# Autodesk Inventor assembly: Outer Shield
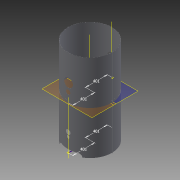
[picture p0: Inventor's stored thumbnail of the model, 180x180]
Saved by Autodesk Inventor 2015 (Build 190159000, 159)
## iProperties
Created: 2014-06-19
Part Number: Outer Shield
Document SubType Name: Assembly
Designer: Aki
Author: Aki
## Documents named in this file (6)
- C:\ColdMatter\CADFiles\EDM Machine\EDM Outer Shield\Outer Shield.iam
- C:\ColdMatter\CADFiles\EDM Machine\EDM Outer Shield\Lower Front Half.ipt
- C:\ColdMatter\CADFiles\EDM Machine\EDM Outer Shield\Lower Back Half.ipt
- C:\ColdMatter\CADFiles\EDM Machine\EDM Outer Shield\Upper Front Half.ipt
- C:\ColdMatter\CADFiles\EDM Machine\EDM Outer Shield\Upper Back Half.ipt
- C:\ColdMatter\CADFiles\EDM Machine\EDM Outer Shield\Band.ipt
## Components (6 placed, 5 different names)
1. Lower Front Half:1 — Mate:1, Mate:2, Mate:3, Mate:4, Mate:5, Mate:7
2. Lower Back Half:1 — Mate:2, Mate:3, Mate:4, Mate:6
3. Upper Front Half:1 — Mate:5, Mate:6, Mate:7, Mate:8, Mate:9, Mate:10, Mate:11
4. Upper Back Half:1 — Mate:8, Mate:9, Mate:10, Mate:12, Mate:13, Mate:15
5. Band:1 — Mate:11, Mate:12, Mate:14
6. Band:2 — Mate:13, Mate:14, Mate:15
## Relationships (15: Mate 15)
- Mate:1: Lower Front Half:1
- Mate:2: Lower Front Half:1 ↔ Lower Back Half:1
- Mate:3: Lower Front Half:1 ↔ Lower Back Half:1
- Mate:4: Lower Front Half:1 ↔ Lower Back Half:1
- Mate:5: Lower Front Half:1 ↔ Upper Front Half:1
- Mate:6: Lower Back Half:1 ↔ Upper Front Half:1
- Mate:7: Lower Front Half:1 ↔ Upper Front Half:1
- Mate:8: Upper Front Half:1 ↔ Upper Back Half:1
- Mate:9: Upper Front Half:1 ↔ Upper Back Half:1
- Mate:10: Upper Front Half:1 ↔ Upper Back Half:1
- Mate:11: Upper Front Half:1 ↔ Band:1
- Mate:12: Upper Back Half:1 ↔ Band:1
- Mate:13: Upper Back Half:1 ↔ Band:2
- Mate:14: Band:1 ↔ Band:2
- Mate:15: Upper Back Half:1 ↔ Band:2
